# Autodesk Inventor assembly: Assembly1
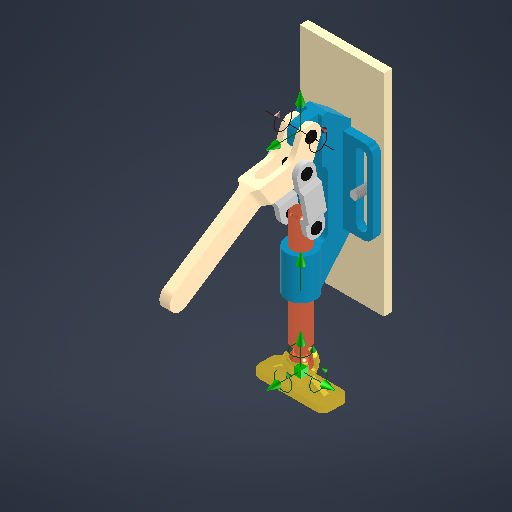
[picture p0: Inventor's stored thumbnail of the model, 512x512]
Saved by Autodesk Inventor 2026 (Build 300175050, 175E)
## iProperties
Created: 2025-05-27
Part Number: Assembly1
Document SubType Name: Assembly
Designer: Saurav Farkade
Author: Saurav Farkade
## Documents named in this file (7)
- C:\Saurav Farkade Windows\Downloads\Assebly+Joints+Exercise+Files\Assembly1.iam
- C:\Saurav Farkade Windows\Downloads\Assebly+Joints+Exercise+Files\FixturePlate.ipt
- C:\Saurav Farkade Windows\Downloads\Assebly+Joints+Exercise+Files\Base_1.ipt
- C:\Saurav Farkade Windows\Downloads\Assebly+Joints+Exercise+Files\Ball_1.ipt
- C:\Saurav Farkade Windows\Downloads\Assebly+Joints+Exercise+Files\Connector_1.ipt
- C:\Saurav Farkade Windows\Downloads\Assebly+Joints+Exercise+Files\Lever_1.ipt
- C:\Saurav Farkade Windows\Downloads\Assebly+Joints+Exercise+Files\Socket_1.ipt
## Components (6 placed, 6 different names)
1. FixturePlate:1 — Slider:2
2. Base_1:1 — Slider:2, Cylindrical:1, Mate:1
3. Ball_1:1 — Cylindrical:1, Rotational:1, Ball:1
4. Connector_1:1 — Rotational:1, Rotational:2
5. Lever_1:1 — Rotational:2, Mate:1
6. Socket_1:1 — Ball:1
## Relationships (6: RevoluteJoint 2, TranslationJoint 1, CylindricalJoint 1, Mate 1, BallJoint 1)
- Slider:2 [TranslationJoint]: FixturePlate:1 ↔ Base_1:1
- Cylindrical:1: Base_1:1 ↔ Ball_1:1
- Rotational:1 [RevoluteJoint]: Ball_1:1 ↔ Connector_1:1
- Rotational:2 [RevoluteJoint]: Connector_1:1 ↔ Lever_1:1
- Mate:1: Base_1:1 ↔ Lever_1:1
- Ball:1: Ball_1:1 ↔ Socket_1:1
